# Autodesk Inventor assembly: linear_cutting_endeffector-3
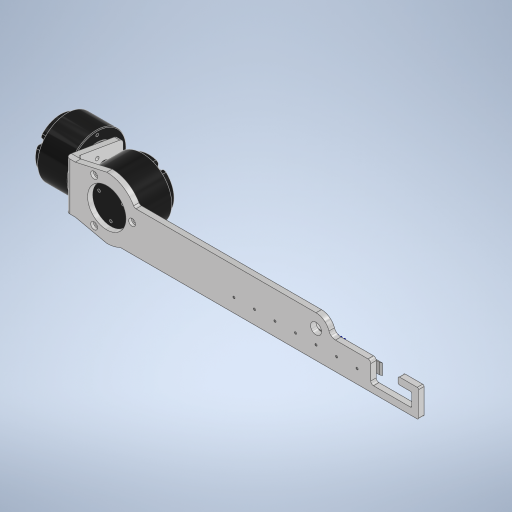
[picture p0: Inventor's stored thumbnail of the model, 512x512]
Saved by Autodesk Inventor 2024 (Build 280153000, 153)
## iProperties
Created: 2025-06-12
Part Number: linear_cutting_endeffector-3
Document SubType Name: Assembly
Designer: 1412z
Author: 1412z
## Documents named in this file (8)
- C:\Users\1412z\OneDrive\デスクトップ\rdclab\harvesting_robot\harvesting_endeffector\linear_cutting_endeffector\linear_cutting_endeffector-3.iam
- C:\Users\1412z\OneDrive\デスクトップ\rdclab\harvesting_robot\harvesting_endeffector\linear_cutting_endeffector\motor_holder\motor_holder-4.ipt
- C:\Users\1412z\OneDrive\デスクトップ\rdclab\harvesting_robot\harvesting_endeffector\linear_cutting_endeffector\misumi\SSE2B6L-100_Autodesk_Inventor_2023_20250607\AIS2023\SSE2B6-100_r.ipt
- C:\Users\1412z\OneDrive\デスクトップ\rdclab\harvesting_robot\harvesting_endeffector\linear_cutting_endeffector\misumi\screw\NBK_SNZSM26\SNZS-M2-6.ipt
- C:\Users\1412z\OneDrive\デスクトップ\rdclab\harvesting_robot\harvesting_endeffector\linear_cutting_endeffector\misumi\SSE2B6L-100_Autodesk_Inventor_2023_20250607\AIS2023\SSEB6_b.ipt
- C:\Users\1412z\OneDrive\デスクトップ\rdclab\harvesting_robot\harvesting_endeffector\linear_cutting_endeffector\misumi\LRGEAM0.8KA-80-K2-B50_Autodesk_Inventor_2024_20250607\LRGEAM0_8KA-80-K2-B50.ipt
- C:\Users\1412z\OneDrive\デスクトップ\rdclab\harvesting_robot\harvesting_endeffector\linear_cutting_endeffector\cutter\pen_type_cutter.ipt
- C:\Users\1412z\OneDrive\デスクトップ\rdclab\harvesting_robot\harvesting_endeffector\linear_cutting_endeffector\GIM3505-08\GIM3505-8_with-driver.ipt
## Components (15 placed, 7 different names)
1. motor_holder-4:1 — 回転:1, 回転:2, 回転:12, 回転:13, 回転:14, 回転:15
2. SSE2B6-100_r:1 — 回転:1, 回転:2, 回転:3, 回転:4, 回転:5, 回転:6, 回転:7, 回転:8, 回転:9, 円柱状:1, 円柱状:2
3. SNZS-M2-6:1 — 回転:3
4. SNZS-M2-6:2 — 回転:4
5. SNZS-M2-6:3 — 回転:5
6. SNZS-M2-6:4 — 回転:6
7. SNZS-M2-6:5 — 回転:7
8. SNZS-M2-6:6 — 回転:8
9. SNZS-M2-6:7 — 回転:9
10. SSEB6_b:1 — 円柱状:1, 回転:10
11. SSEB6_b:2 — 円柱状:2, 回転:11
12. LRGEAM0_8KA-80-K2-B50:1 — 回転:10, 回転:11
13. pen_type_cutter:1
14. GIM3505-8_with-driver:1 — 回転:12, 回転:13
15. GIM3505-8_with-driver:2 — 回転:14, 回転:15
## Relationships (17: RevoluteJoint 15, CylindricalJoint 2)
- 回転:1 [RevoluteJoint]: motor_holder-4:1 ↔ SSE2B6-100_r:1
- 回転:2 [RevoluteJoint]: motor_holder-4:1 ↔ SSE2B6-100_r:1
- 回転:3 [RevoluteJoint]: SSE2B6-100_r:1 ↔ SNZS-M2-6:1
- 回転:4 [RevoluteJoint]: SSE2B6-100_r:1 ↔ SNZS-M2-6:2
- 回転:5 [RevoluteJoint]: SSE2B6-100_r:1 ↔ SNZS-M2-6:3
- 回転:6 [RevoluteJoint]: SSE2B6-100_r:1 ↔ SNZS-M2-6:4
- 回転:7 [RevoluteJoint]: SSE2B6-100_r:1 ↔ SNZS-M2-6:5
- 回転:8 [RevoluteJoint]: SSE2B6-100_r:1 ↔ SNZS-M2-6:6
- 回転:9 [RevoluteJoint]: SSE2B6-100_r:1 ↔ SNZS-M2-6:7
- 円柱状:1 [CylindricalJoint]: SSE2B6-100_r:1 ↔ SSEB6_b:1
- 円柱状:2 [CylindricalJoint]: SSE2B6-100_r:1 ↔ SSEB6_b:2
- 回転:10 [RevoluteJoint]: SSEB6_b:1 ↔ LRGEAM0_8KA-80-K2-B50:1
- 回転:11 [RevoluteJoint]: SSEB6_b:2 ↔ LRGEAM0_8KA-80-K2-B50:1
- 回転:12 [RevoluteJoint]: motor_holder-4:1 ↔ GIM3505-8_with-driver:1
- 回転:13 [RevoluteJoint]: motor_holder-4:1 ↔ GIM3505-8_with-driver:1
- 回転:14 [RevoluteJoint]: motor_holder-4:1 ↔ GIM3505-8_with-driver:2
- 回転:15 [RevoluteJoint]: motor_holder-4:1 ↔ GIM3505-8_with-driver:2
